# Autodesk Inventor assembly: Main Assembly
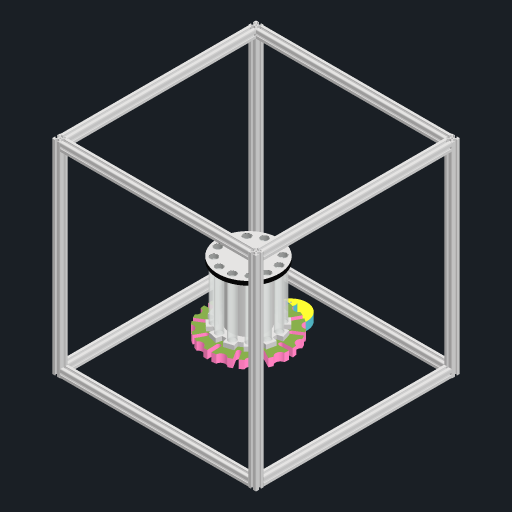
[picture p0: Inventor's stored thumbnail of the model, 512x512]
Saved by Autodesk Inventor 2023.1 (Build 271208000, 208)
## iProperties
Created: 2022-10-27
Part Number: Main Assembly
Document SubType Name: Assembly
Designer: JARRETT
Author: JARRETT
## Documents named in this file (5)
- C:\Users\Jarrett\Desktop\Projects\BehrendURCMechanical\CAD\Science\Main Assembly.iam
- C:\Users\Jarrett\Desktop\Projects\BehrendURCMechanical\CAD\Science\8020 Frame Horizontal.ipt
- C:\Users\Jarrett\Desktop\Projects\BehrendURCMechanical\CAD\Science\8020 Frame Vertical.ipt
- C:\Users\Jarrett\Desktop\Projects\BehrendURCMechanical\CAD\Science\12 Geneva Assembly.iam
- C:\Users\Jarrett\Desktop\Projects\BehrendURCMechanical\CAD\Science\Test Tube.ipt
## Components (25 placed, 4 different names)
1. 8020 Frame Horizontal:1 — Rigid:1, Rigid:2
2. 8020 Frame Vertical:1 — Rigid:1, Rigid:9
3. 8020 Frame Vertical:2 — Rigid:2, Rigid:3, Rigid:10
4. 8020 Frame Vertical:3 — Rigid:4, Rigid:5
5. 8020 Frame Vertical:4 — Rigid:6, Rigid:7, Rigid:8, Rigid:11
6. 8020 Frame Horizontal:2 — Rigid:7
7. 8020 Frame Horizontal:3 — Rigid:3, Rigid:4
8. 8020 Frame Horizontal:4 — Rigid:5, Rigid:6
9. 8020 Frame Horizontal:5 — Rigid:8
10. 8020 Frame Horizontal:6 — Rigid:9
11. 8020 Frame Horizontal:7 — Rigid:10
12. 8020 Frame Horizontal:8 — Rigid:11
13. 12 Geneva Assembly:1 [sub-assembly] — Mate:1, Tangent:1
14. Test Tube:1 — Mate:1, Tangent:1
15. Test Tube:2
16. Test Tube:3
17. Test Tube:4
18. Test Tube:5
19. Test Tube:6
20. Test Tube:7
21. Test Tube:8
22. Test Tube:9
23. Test Tube:10
24. Test Tube:11
25. Test Tube:12
## Component patterns: (12 elements, first: Test Tube:1)
## Relationships (13: WeldJoint 11, Mate 1, Tangent 1)
- Rigid:1 [WeldJoint]: 8020 Frame Horizontal:1 ↔ 8020 Frame Vertical:1
- Rigid:2 [WeldJoint]: 8020 Frame Horizontal:1 ↔ 8020 Frame Vertical:2
- Rigid:3 [WeldJoint]: 8020 Frame Vertical:2 ↔ 8020 Frame Horizontal:3
- Rigid:4 [WeldJoint]: 8020 Frame Vertical:3 ↔ 8020 Frame Horizontal:3
- Rigid:5 [WeldJoint]: 8020 Frame Vertical:3 ↔ 8020 Frame Horizontal:4
- Rigid:6 [WeldJoint]: 8020 Frame Vertical:4 ↔ 8020 Frame Horizontal:4
- Rigid:7 [WeldJoint]: 8020 Frame Vertical:4 ↔ 8020 Frame Horizontal:2
- Rigid:8 [WeldJoint]: 8020 Frame Vertical:4 ↔ 8020 Frame Horizontal:5
- Rigid:9 [WeldJoint]: 8020 Frame Vertical:1 ↔ 8020 Frame Horizontal:6
- Rigid:10 [WeldJoint]: 8020 Frame Vertical:2 ↔ 8020 Frame Horizontal:7
- Rigid:11 [WeldJoint]: 8020 Frame Vertical:4 ↔ 8020 Frame Horizontal:8
- Mate:1: 12 Geneva Assembly:1 ↔ Test Tube:1
- Tangent:1: 12 Geneva Assembly:1 ↔ Test Tube:1
